# Autodesk Inventor assembly: leg_assembly
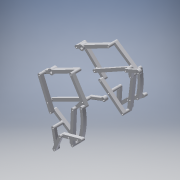
[picture p0: Inventor's stored thumbnail of the model, 180x180]
Saved by Autodesk Inventor 2017 (Build 210142000, 142)
## iProperties
Created: 2021-01-25
Part Number: leg_assembly
Document SubType Name: Assembly
Designer: agustin
Author: agustin
## Documents named in this file (23)
- D:\Agustin\Mis proyectos\Mechanisms\WalkingRobot\leg_assembly.iam
- D:\Agustin\Mis proyectos\Mechanisms\WalkingRobot\bone0.ipt
- D:\Agustin\Mis proyectos\Mechanisms\WalkingRobot\bone1.ipt
- D:\Agustin\Mis proyectos\Mechanisms\WalkingRobot\bone2.ipt
- D:\Agustin\Mis proyectos\Mechanisms\WalkingRobot\bone3.ipt
- D:\Agustin\Mis proyectos\Mechanisms\WalkingRobot\bone4.ipt
- D:\Agustin\Mis proyectos\Mechanisms\WalkingRobot\bone5.ipt
- D:\Agustin\Mis proyectos\Mechanisms\WalkingRobot\bone6.ipt
- D:\Agustin\Mis proyectos\Mechanisms\WalkingRobot\bone7.ipt
- D:\Agustin\Mis proyectos\Mechanisms\WalkingRobot\base-bone.ipt
- D:\Agustin\Mis proyectos\Mechanisms\WalkingRobot\toe1.ipt
- D:\Agustin\Mis proyectos\Mechanisms\WalkingRobot\toe2.ipt
- D:\Agustin\Mis proyectos\Mechanisms\WalkingRobot\bone0_MIR.ipt
- D:\Agustin\Mis proyectos\Mechanisms\WalkingRobot\bone1_MIR.ipt
- D:\Agustin\Mis proyectos\Mechanisms\WalkingRobot\bone2_MIR.ipt
- D:\Agustin\Mis proyectos\Mechanisms\WalkingRobot\bone3_MIR.ipt
- D:\Agustin\Mis proyectos\Mechanisms\WalkingRobot\bone4_MIR.ipt
- D:\Agustin\Mis proyectos\Mechanisms\WalkingRobot\bone5_MIR.ipt
- D:\Agustin\Mis proyectos\Mechanisms\WalkingRobot\bone7_MIR.ipt
- D:\Agustin\Mis proyectos\Mechanisms\WalkingRobot\base-bone_MIR.ipt
- D:\Agustin\Mis proyectos\Mechanisms\WalkingRobot\toe1_MIR.ipt
- D:\Agustin\Mis proyectos\Mechanisms\WalkingRobot\toe2_MIR.ipt
- D:\Agustin\Mis proyectos\Mechanisms\WalkingRobot\bone6_MIR.ipt
## Components (22 placed, 22 different names)
1. bone0:1 — Mate:12, Mate:13, Mate:14, Mate:15
2. bone1:1 — Mate:7, Mate:9, Mate:10, Mate:19
3. bone2:1 — Mate:5, Mate:6, Mate:8, Mate:11
4. bone3:1 — Mate:8, Mate:9, Mate:11, Mate:24
5. bone4:1 — Mate:17, Mate:18, Mate:19, Mate:20, Mate:21
6. bone5:1 — Mate:13, Mate:15, Mate:16, Mate:17, Mate:18
7. bone7:1 — Mate:1, Mate:2, Mate:3, Mate:4, Mate:16
8. base-bone:1 — Mate:1, Mate:4, Mate:5, Mate:6, Mate:7, Mate:10, Mate:12, Mate:14
9. toe1:1 — Mate:20, Mate:21, Mate:22, Mate:23
10. toe2:1 — Mate:22, Mate:23, Mate:24
11. bone6:2 — Mate:2, Mate:3
12. bone0_MIR:1 — Mate:31, Mate:32, Mate:34, Mate:35
13. bone1_MIR:1 — Mate:26, Mate:28, Mate:36, Mate:37
14. bone2_MIR:1 — Mate:25, Mate:27, Mate:38, Mate:39
15. bone3_MIR:1 — Mate:25, Mate:26, Mate:27, Mate:44
16. bone4_MIR:1 — Mate:28, Mate:29, Mate:30, Mate:42, Mate:43
17. bone5_MIR:1 — Mate:29, Mate:30, Mate:31, Mate:32, Mate:33
18. bone7_MIR:1 — Mate:33, Mate:40, Mate:41, Mate:47, Mate:48
19. base-bone_MIR:1 — Mate:34, Mate:35, Mate:36, Mate:37, Mate:38, Mate:39, Mate:40, Mate:41
20. toe1_MIR:1 — Mate:42, Mate:43, Mate:45, Mate:46
21. toe2_MIR:1 — Mate:44, Mate:45, Mate:46
22. bone6_MIR:1 — Mate:47, Mate:48
## Relationships (48: Mate 48)
- Mate:1: bone7:1 ↔ base-bone:1
- Mate:2: bone7:1 ↔ bone6:2
- Mate:3: bone7:1 ↔ bone6:2
- Mate:4: bone7:1 ↔ base-bone:1
- Mate:5: bone2:1 ↔ base-bone:1
- Mate:6: bone2:1 ↔ base-bone:1
- Mate:7: bone1:1 ↔ base-bone:1
- Mate:8: bone2:1 ↔ bone3:1
- Mate:9: bone1:1 ↔ bone3:1
- Mate:10: bone1:1 ↔ base-bone:1
- Mate:11: bone2:1 ↔ bone3:1
- Mate:12: bone0:1 ↔ base-bone:1
- Mate:13: bone0:1 ↔ bone5:1
- Mate:14: bone0:1 ↔ base-bone:1
- Mate:15: bone0:1 ↔ bone5:1
- Mate:16: bone5:1 ↔ bone7:1
- Mate:17: bone4:1 ↔ bone5:1
- Mate:18: bone4:1 ↔ bone5:1
- Mate:19: bone1:1 ↔ bone4:1
- Mate:20: bone4:1 ↔ toe1:1
- Mate:21: bone4:1 ↔ toe1:1
- Mate:22: toe1:1 ↔ toe2:1
- Mate:23: toe1:1 ↔ toe2:1
- Mate:24: bone3:1 ↔ toe2:1
- Mate:25: bone2_MIR:1 ↔ bone3_MIR:1
- Mate:26: bone1_MIR:1 ↔ bone3_MIR:1
- Mate:27: bone2_MIR:1 ↔ bone3_MIR:1
- Mate:28: bone1_MIR:1 ↔ bone4_MIR:1
- Mate:29: bone4_MIR:1 ↔ bone5_MIR:1
- Mate:30: bone4_MIR:1 ↔ bone5_MIR:1
- Mate:31: bone0_MIR:1 ↔ bone5_MIR:1
- Mate:32: bone0_MIR:1 ↔ bone5_MIR:1
- Mate:33: bone5_MIR:1 ↔ bone7_MIR:1
- Mate:34: bone0_MIR:1 ↔ base-bone_MIR:1
- Mate:35: bone0_MIR:1 ↔ base-bone_MIR:1
- Mate:36: bone1_MIR:1 ↔ base-bone_MIR:1
- Mate:37: bone1_MIR:1 ↔ base-bone_MIR:1
- Mate:38: bone2_MIR:1 ↔ base-bone_MIR:1
- Mate:39: bone2_MIR:1 ↔ base-bone_MIR:1
- Mate:40: bone7_MIR:1 ↔ base-bone_MIR:1
- Mate:41: bone7_MIR:1 ↔ base-bone_MIR:1
- Mate:42: bone4_MIR:1 ↔ toe1_MIR:1
- Mate:43: bone4_MIR:1 ↔ toe1_MIR:1
- Mate:44: bone3_MIR:1 ↔ toe2_MIR:1
- Mate:45: toe1_MIR:1 ↔ toe2_MIR:1
- Mate:46: toe1_MIR:1 ↔ toe2_MIR:1
- Mate:47: bone7_MIR:1 ↔ bone6_MIR:1
- Mate:48: bone7_MIR:1 ↔ bone6_MIR:1
